# Autodesk Inventor assembly: Plate Assembly
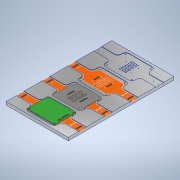
[picture p0: Inventor's stored thumbnail of the model, 180x180]
Saved by Autodesk Inventor 2022 (Build 260153000, 153)
## iProperties
Created: 2021-07-16
Part Number: Plate Assembly
Document SubType Name: Assembly
Designer: Caleb
Author: Caleb
## Documents named in this file (7)
- C:\Users\Caleb\Desktop\nebraska-silicon-lab\Hardware\ETL\Module Assembly\Tamale Assembly Plate V1\Plate Assembly.iam
- C:\Users\Caleb\Desktop\nebraska-silicon-lab\Hardware\ETL\Module Assembly\Tamale Assembly Plate V1\Tamale Assembly Plate.ipt
- C:\Users\Caleb\Desktop\nebraska-silicon-lab\Hardware\ETL\Module Assembly\Tamale Assembly Plate V1\Flex Assembly.iam
- C:\Users\Caleb\Desktop\nebraska-silicon-lab\Hardware\ETL\Module Assembly\Tamale Assembly Plate V1\spacer.ipt
- C:\Users\Caleb\Desktop\nebraska-silicon-lab\Hardware\ETL\Module Assembly\Tamale Assembly Plate V1\90910A443_BUTTON HEAD TORX SCREWS.ipt
- C:\Users\Caleb\Desktop\nebraska-silicon-lab\Hardware\ETL\Module Assembly\Tamale Assembly Plate V1\Mock Module PCB.iam
- C:\Users\Caleb\Desktop\nebraska-silicon-lab\Hardware\ETL\Module Assembly\Tamale Assembly Plate V1\91585A353_18-8 STAINLESS STEEL DOWEL PIN.ipt
## Components (43 placed, 6 different names)
1. Tamale Assembly Plate:1 — Mate:1, Mate:2, Mate:3, Flush:1, Flush:2, Flush:3, Mate:6, Mate:7, Insert:1, Mate:10, Mate:11, Insert:7, Insert:12, Insert:13, Insert:14, Insert:15, Insert:16, Insert:17, Insert:18, Insert:19, Insert:20, Insert:21, Insert:22, Insert:23, Insert:24
2. Flex Assembly:1 [sub-assembly] — Mate:2, Flush:2, Mate:9, Insert:7, Insert:25, Insert:26, Insert:27, Insert:28, Insert:37, Insert:38, Insert:39, Insert:40
3. Flex Assembly:2 [sub-assembly] — Mate:3, Flush:3, Insert:20, Insert:29, Insert:30, Insert:31, Insert:32, Insert:33, Insert:34, Insert:35, Insert:36
4. Flex Assembly:4 [sub-assembly] — Mate:1, Flush:1, Mate:5, Insert:1, Insert:2, Insert:3, Insert:4, Insert:5, Insert:41, Insert:42, Insert:43, Insert:44
5. spacer:1 — Mate:5, Mate:6, Mate:7, Mate:8, Angle:1, Insert:6
6. 90910A443_BUTTON HEAD TORX SCREWS:1 — Insert:2
7. 90910A443_BUTTON HEAD TORX SCREWS:2 — Insert:3
8. 90910A443_BUTTON HEAD TORX SCREWS:3 — Insert:5
9. 90910A443_BUTTON HEAD TORX SCREWS:4 — Insert:4
10. Mock Module PCB:1 [sub-assembly] — Mate:8, Angle:1, Insert:6
11. spacer:2 — Mate:9, Mate:10, Mate:11
12. 91585A353_18-8 STAINLESS STEEL DOWEL PIN:1 — Insert:12
13. 91585A353_18-8 STAINLESS STEEL DOWEL PIN:2 — Insert:13
14. 91585A353_18-8 STAINLESS STEEL DOWEL PIN:3 — Insert:14
15. 91585A353_18-8 STAINLESS STEEL DOWEL PIN:4 — Insert:15
16. 91585A353_18-8 STAINLESS STEEL DOWEL PIN:5 — Insert:16
17. 91585A353_18-8 STAINLESS STEEL DOWEL PIN:6 — Insert:17
18. 91585A353_18-8 STAINLESS STEEL DOWEL PIN:7 — Insert:18
19. 91585A353_18-8 STAINLESS STEEL DOWEL PIN:8 — Insert:19
20. 91585A353_18-8 STAINLESS STEEL DOWEL PIN:9 — Insert:21
21. 91585A353_18-8 STAINLESS STEEL DOWEL PIN:10 — Insert:22
22. 91585A353_18-8 STAINLESS STEEL DOWEL PIN:11 — Insert:23
23. 91585A353_18-8 STAINLESS STEEL DOWEL PIN:12 — Insert:24
24. 90910A443_BUTTON HEAD TORX SCREWS:5 — Insert:25
25. 90910A443_BUTTON HEAD TORX SCREWS:6 — Insert:26
26. 90910A443_BUTTON HEAD TORX SCREWS:7 — Insert:28
27. 90910A443_BUTTON HEAD TORX SCREWS:8 — Insert:27
28. 90910A443_BUTTON HEAD TORX SCREWS:9 — Insert:29
29. 90910A443_BUTTON HEAD TORX SCREWS:10 — Insert:31
30. 90910A443_BUTTON HEAD TORX SCREWS:11 — Insert:32
31. 90910A443_BUTTON HEAD TORX SCREWS:12 — Insert:30
32. 90910A443_BUTTON HEAD TORX SCREWS:13 — Insert:33
33. 90910A443_BUTTON HEAD TORX SCREWS:14 — Insert:34
34. 90910A443_BUTTON HEAD TORX SCREWS:15 — Insert:35
35. 90910A443_BUTTON HEAD TORX SCREWS:16 — Insert:36
36. 90910A443_BUTTON HEAD TORX SCREWS:17 — Insert:40
37. 90910A443_BUTTON HEAD TORX SCREWS:18 — Insert:39
38. 90910A443_BUTTON HEAD TORX SCREWS:19 — Insert:38
39. 90910A443_BUTTON HEAD TORX SCREWS:20 — Insert:37
40. 90910A443_BUTTON HEAD TORX SCREWS:21 — Insert:43
41. 90910A443_BUTTON HEAD TORX SCREWS:22 — Insert:44
42. 90910A443_BUTTON HEAD TORX SCREWS:23 — Insert:41
43. 90910A443_BUTTON HEAD TORX SCREWS:24 — Insert:42
## Relationships (54: Insert 40, Mate 10, Flush 3, Angle 1)
- Mate:1: Tamale Assembly Plate:1 ↔ Flex Assembly:4
- Mate:2: Tamale Assembly Plate:1 ↔ Flex Assembly:1
- Mate:3: Tamale Assembly Plate:1 ↔ Flex Assembly:2
- Flush:1: Tamale Assembly Plate:1 ↔ Flex Assembly:4
- Flush:2: Tamale Assembly Plate:1 ↔ Flex Assembly:1
- Flush:3: Tamale Assembly Plate:1 ↔ Flex Assembly:2
- Mate:5: Flex Assembly:4 ↔ spacer:1
- Mate:6: Tamale Assembly Plate:1 ↔ spacer:1
- Mate:7: Tamale Assembly Plate:1 ↔ spacer:1
- Insert:1: Tamale Assembly Plate:1 ↔ Flex Assembly:4
- Insert:2: Flex Assembly:4 ↔ 90910A443_BUTTON HEAD TORX SCREWS:1
- Insert:3: Flex Assembly:4 ↔ 90910A443_BUTTON HEAD TORX SCREWS:2
- Insert:4: Flex Assembly:4 ↔ 90910A443_BUTTON HEAD TORX SCREWS:4
- Insert:5: Flex Assembly:4 ↔ 90910A443_BUTTON HEAD TORX SCREWS:3
- Mate:8: spacer:1 ↔ Mock Module PCB:1
- Angle:1 (0 deg): spacer:1 ↔ Mock Module PCB:1
- Insert:6: spacer:1 ↔ Mock Module PCB:1
- Mate:9: Flex Assembly:1 ↔ spacer:2
- Mate:10: Tamale Assembly Plate:1 ↔ spacer:2
- Mate:11: Tamale Assembly Plate:1 ↔ spacer:2
- Insert:7: Tamale Assembly Plate:1 ↔ Flex Assembly:1
- Insert:12: Tamale Assembly Plate:1 ↔ 91585A353_18-8 STAINLESS STEEL DOWEL PIN:1
- Insert:13: Tamale Assembly Plate:1 ↔ 91585A353_18-8 STAINLESS STEEL DOWEL PIN:2
- Insert:14: Tamale Assembly Plate:1 ↔ 91585A353_18-8 STAINLESS STEEL DOWEL PIN:3
- Insert:15: Tamale Assembly Plate:1 ↔ 91585A353_18-8 STAINLESS STEEL DOWEL PIN:4
- Insert:16: Tamale Assembly Plate:1 ↔ 91585A353_18-8 STAINLESS STEEL DOWEL PIN:5
- Insert:17: Tamale Assembly Plate:1 ↔ 91585A353_18-8 STAINLESS STEEL DOWEL PIN:6
- Insert:18: Tamale Assembly Plate:1 ↔ 91585A353_18-8 STAINLESS STEEL DOWEL PIN:7
- Insert:19: Tamale Assembly Plate:1 ↔ 91585A353_18-8 STAINLESS STEEL DOWEL PIN:8
- Insert:20: Tamale Assembly Plate:1 ↔ Flex Assembly:2
- Insert:21: Tamale Assembly Plate:1 ↔ 91585A353_18-8 STAINLESS STEEL DOWEL PIN:9
- Insert:22: Tamale Assembly Plate:1 ↔ 91585A353_18-8 STAINLESS STEEL DOWEL PIN:10
- Insert:23: Tamale Assembly Plate:1 ↔ 91585A353_18-8 STAINLESS STEEL DOWEL PIN:11
- Insert:24: Tamale Assembly Plate:1 ↔ 91585A353_18-8 STAINLESS STEEL DOWEL PIN:12
- Insert:25: Flex Assembly:1 ↔ 90910A443_BUTTON HEAD TORX SCREWS:5
- Insert:26: Flex Assembly:1 ↔ 90910A443_BUTTON HEAD TORX SCREWS:6
- Insert:27: Flex Assembly:1 ↔ 90910A443_BUTTON HEAD TORX SCREWS:8
- Insert:28: Flex Assembly:1 ↔ 90910A443_BUTTON HEAD TORX SCREWS:7
- Insert:29: Flex Assembly:2 ↔ 90910A443_BUTTON HEAD TORX SCREWS:9
- Insert:30: Flex Assembly:2 ↔ 90910A443_BUTTON HEAD TORX SCREWS:12
- Insert:31: Flex Assembly:2 ↔ 90910A443_BUTTON HEAD TORX SCREWS:10
- Insert:32: Flex Assembly:2 ↔ 90910A443_BUTTON HEAD TORX SCREWS:11
- Insert:33: Flex Assembly:2 ↔ 90910A443_BUTTON HEAD TORX SCREWS:13
- Insert:34: Flex Assembly:2 ↔ 90910A443_BUTTON HEAD TORX SCREWS:14
- Insert:35: Flex Assembly:2 ↔ 90910A443_BUTTON HEAD TORX SCREWS:15
- Insert:36: Flex Assembly:2 ↔ 90910A443_BUTTON HEAD TORX SCREWS:16
- Insert:37: Flex Assembly:1 ↔ 90910A443_BUTTON HEAD TORX SCREWS:20
- Insert:38: Flex Assembly:1 ↔ 90910A443_BUTTON HEAD TORX SCREWS:19
- Insert:39: Flex Assembly:1 ↔ 90910A443_BUTTON HEAD TORX SCREWS:18
- Insert:40: Flex Assembly:1 ↔ 90910A443_BUTTON HEAD TORX SCREWS:17
- Insert:41: Flex Assembly:4 ↔ 90910A443_BUTTON HEAD TORX SCREWS:23
- Insert:42: Flex Assembly:4 ↔ 90910A443_BUTTON HEAD TORX SCREWS:24
- Insert:43: Flex Assembly:4 ↔ 90910A443_BUTTON HEAD TORX SCREWS:21
- Insert:44: Flex Assembly:4 ↔ 90910A443_BUTTON HEAD TORX SCREWS:22
